# Autodesk Inventor assembly: A2017_T5_05
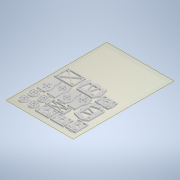
[picture p0: Inventor's stored thumbnail of the model, 180x180]
Saved by Autodesk Inventor 2020 (Build 240168000, 168)
## iProperties
Created: 2021-08-27
Part Number: A2017_T5_05
Document SubType Name: Assembly
Designer: Masato
Author: Masato
## Documents named in this file (8)
- D:\GitHub\inventor\SUSTAINA-OP\Cam\A2017_T5_05.iam
- D:\GitHub\inventor\SUSTAINA-OP\Cam\DisposableBoard.ipt
- D:\GitHub\inventor\SUSTAINA-OP\UpperBody\Trunk\CrossRollerBearing\Inner_support_stand.ipt
- D:\GitHub\inventor\SUSTAINA-OP\LowerBody\Leg_joint\Leg_joint_yaw_frame.ipt
- D:\GitHub\inventor\SUSTAINA-OP\LowerBody\Link\BackLink_diagonal.ipt
- D:\GitHub\inventor\SUSTAINA-OP\LowerBody\Link\FrontLink_diagonal.ipt
- D:\GitHub\inventor\SUSTAINA-OP\UpperBody\Arm\Shoulder_horn_frame.ipt
- D:\GitHub\inventor\SUSTAINA-OP\UpperBody\Trunk\Trunk_lower_side_frame.ipt
## Components (17 placed, 7 different names)
1. DisposableBoard:1 — メイト:2, メイト:1, フラッシュ:1, フラッシュ:2, メイト:20, 角度:4, 正接:1, 正接:2, メイト:21, メイト:22, メイト:24, メイト:25, 正接:4, 角度:5, メイト:26, フラッシュ:5, メイト:28, メイト:29, 角度:6, フラッシュ:8, メイト:32, メイト:33, 角度:7
2. FrontLink_diagonal:1 — メイト:22, メイト:31, フラッシュ:8, フラッシュ:9, 正接:10
3. BackLink_diagonal:1 — メイト:21, メイト:27, フラッシュ:6
4. Shoulder_horn_frame:3 — メイト:28, フラッシュ:7, メイト:30, 正接:8
5. Trunk_lower_side_frame:1 — メイト:29, 角度:6, 正接:8, 正接:9, 正接:11
6. Trunk_lower_side_frame:2 — メイト:32, フラッシュ:9, 正接:10, 正接:12
7. Shoulder_horn_frame:4 — メイト:33, 角度:7, 正接:11, 正接:12
8. Inner_support_stand:1 — メイト:20, 角度:4, 正接:1, 正接:2
9. Inner_support_stand:2 — 正接:7
10. Inner_support_stand:3 — 正接:5
11. Inner_support_stand:4
12. Leg_joint_yaw_frame:1 — メイト:24, 正接:4, 角度:5, 正接:5, フラッシュ:4, 正接:6, メイト:31
13. Leg_joint_yaw_frame:2 — メイト:25, フラッシュ:4, 正接:6
14. Leg_joint_yaw_frame:3
15. Leg_joint_yaw_frame:4 — 正接:9
16. Shoulder_horn_frame:1 — メイト:26, フラッシュ:5, 正接:7, メイト:27, フラッシュ:6
17. Shoulder_horn_frame:2 — フラッシュ:7, メイト:30
## Component patterns: (4 elements, first: Inner_support_stand:1), (2 elements, first: Leg_joint_yaw_frame:1 + Leg_joint_yaw_frame:2), (2 elements, first: Shoulder_horn_frame:1)
## Relationships (38: Mate 15, Tangent 11, Flush 8, Angle 4)
- メイト:2 [Mate]: DisposableBoard:1
- メイト:1 [Mate]: DisposableBoard:1
- フラッシュ:1 [Flush]: DisposableBoard:1
- フラッシュ:2 [Flush]: DisposableBoard:1
- メイト:20 [Mate]: DisposableBoard:1 ↔ Inner_support_stand:1
- 角度:4 [Angle] (0 deg): DisposableBoard:1 ↔ Inner_support_stand:1
- 正接:1 [Tangent] (2 mm): DisposableBoard:1 ↔ Inner_support_stand:1
- 正接:2 [Tangent] (2 mm): DisposableBoard:1 ↔ Inner_support_stand:1
- メイト:21 [Mate]: DisposableBoard:1 ↔ BackLink_diagonal:1
- メイト:22 [Mate]: DisposableBoard:1 ↔ FrontLink_diagonal:1
- メイト:24 [Mate]: DisposableBoard:1 ↔ Leg_joint_yaw_frame:1
- メイト:25 [Mate]: DisposableBoard:1 ↔ Leg_joint_yaw_frame:2
- 正接:4 [Tangent] (2 mm): DisposableBoard:1 ↔ Leg_joint_yaw_frame:1
- 角度:5 [Angle] (0 deg): DisposableBoard:1 ↔ Leg_joint_yaw_frame:1
- 正接:5 [Tangent] (2.5 mm): Inner_support_stand:3 ↔ Leg_joint_yaw_frame:1
- フラッシュ:4 [Flush]: Leg_joint_yaw_frame:1 ↔ Leg_joint_yaw_frame:2
- 正接:6 [Tangent] (3 mm): Leg_joint_yaw_frame:1 ↔ Leg_joint_yaw_frame:2
- メイト:26 [Mate]: DisposableBoard:1 ↔ Shoulder_horn_frame:1
- フラッシュ:5 [Flush] (2 mm): DisposableBoard:1 ↔ Shoulder_horn_frame:1
- 正接:7 [Tangent] (2.5 mm): Inner_support_stand:2 ↔ Shoulder_horn_frame:1
- メイト:27 [Mate] (2.5 mm): BackLink_diagonal:1 ↔ Shoulder_horn_frame:1
- フラッシュ:6 [Flush]: BackLink_diagonal:1 ↔ Shoulder_horn_frame:1
- メイト:28 [Mate]: DisposableBoard:1 ↔ Shoulder_horn_frame:3
- メイト:29 [Mate]: DisposableBoard:1 ↔ Trunk_lower_side_frame:1
- フラッシュ:7 [Flush]: Shoulder_horn_frame:3 ↔ Shoulder_horn_frame:2
- メイト:30 [Mate] (2.5 mm): Shoulder_horn_frame:3 ↔ Shoulder_horn_frame:2
- 角度:6 [Angle] (90 deg): DisposableBoard:1 ↔ Trunk_lower_side_frame:1
- 正接:8 [Tangent] (2.5 mm): Shoulder_horn_frame:3 ↔ Trunk_lower_side_frame:1
- 正接:9 [Tangent] (2.5 mm): Trunk_lower_side_frame:1 ↔ Leg_joint_yaw_frame:4
- メイト:31 [Mate] (2.5 mm): FrontLink_diagonal:1 ↔ Leg_joint_yaw_frame:1
- フラッシュ:8 [Flush] (2 mm): DisposableBoard:1 ↔ FrontLink_diagonal:1
- メイト:32 [Mate]: DisposableBoard:1 ↔ Trunk_lower_side_frame:2
- フラッシュ:9 [Flush]: FrontLink_diagonal:1 ↔ Trunk_lower_side_frame:2
- 正接:10 [Tangent] (2.5 mm): FrontLink_diagonal:1 ↔ Trunk_lower_side_frame:2
- メイト:33 [Mate]: DisposableBoard:1 ↔ Shoulder_horn_frame:4
- 角度:7 [Angle] (0 deg): DisposableBoard:1 ↔ Shoulder_horn_frame:4
- 正接:11 [Tangent] (2.5 mm): Trunk_lower_side_frame:1 ↔ Shoulder_horn_frame:4
- 正接:12 [Tangent] (2.5 mm): Trunk_lower_side_frame:2 ↔ Shoulder_horn_frame:4
